# Autodesk Inventor assembly: Assembly1
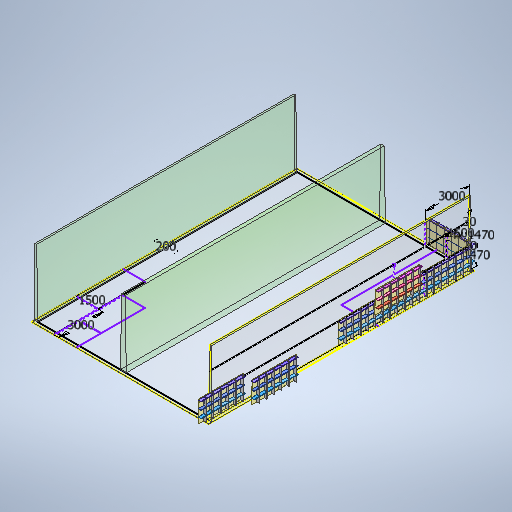
[picture p0: Inventor's stored thumbnail of the model, 512x512]
Saved by Autodesk Inventor 2026.2 (Build 302298000, 298)
## iProperties
Created: 2026-04-17
Part Number: Assembly1
Document SubType Name: Assembly
Designer: admin
Author: admin
## Documents named in this file (4)
- C:\Users\admin\Documents\Inventor\GBK-Gubkinskiy\Assembly1.iam
- C:\Users\admin\Documents\Inventor\GBK-Gubkinskiy\Part1.ipt
- C:\Users\admin\Documents\Inventor\GBK-Gubkinskiy\Assembly shield 1.iam
- C:\Users\admin\Documents\Inventor\GBK-Gubkinskiy\Assembly shield 1_CPY2.iam
## Components (8 placed, 3 different names)
1. Part1:1 — Mate:9
2. Assembly shield 1:1 [sub-assembly]
3. Assembly shield 1_CPY2:1 [sub-assembly]
4. Assembly shield 1:2 [sub-assembly]
5. Assembly shield 1:3 [sub-assembly]
6. Assembly shield 1:4 [sub-assembly] — Mate:9
7. Assembly shield 1:5 [sub-assembly]
8. Assembly shield 1:6 [sub-assembly]
## Relationships (3: Mate 2, Flush 1)
- [Flush]: Part1:1 ↔ Assembly shield 1:1
- [Mate]: Part1:1 ↔ Assembly shield 1:1
- Mate:9: Part1:1 ↔ Assembly shield 1:4
